# Autodesk Inventor assembly: karikumi
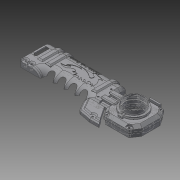
[picture p0: Inventor's stored thumbnail of the model, 180x180]
Saved by Autodesk Inventor 2018 (Build 220112000, 112)
## iProperties
Created: 2019-02-27
Part Number: karikumi
Material: 一般
Document SubType Name: Assembly
Designer: ku_sk
Author: ku_sk
## Documents named in this file (3)
- E:\windows\InventorProjects\BayBladeLauncher\type2\karikumi.iam
- E:\windows\InventorProjects\BayBladeLauncher\type2\parts\conectcover.ipt
- E:\windows\InventorProjects\BayBladeLauncher\type2\parts\undercover.ipt
## Components (2 placed, 2 different names)
1. conectcover:1 — メイト:4, メイト:6
2. undercover:1 — メイト:1, メイト:2, メイト:3, メイト:4, メイト:6
## Relationships (5: Mate 5)
- メイト:1 [Mate]: undercover:1
- メイト:2 [Mate]: undercover:1
- メイト:3 [Mate]: undercover:1
- メイト:4 [Mate]: conectcover:1 ↔ undercover:1
- メイト:6 [Mate]: conectcover:1 ↔ undercover:1
